# Autodesk Inventor assembly: TourniquetPCBV1_Updated
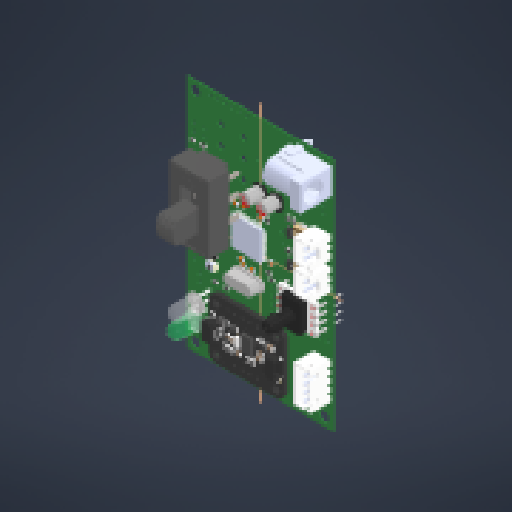
[picture p0: Inventor's stored thumbnail of the model, 512x512]
Saved by Autodesk Inventor 2026.2 (Build 302298010, 298A)
## iProperties
Company: Open CASCADE
Created: 2026-02-03
Part Number: TourniquetPCBV1_Updated
Description: Open CASCADE Model
Document SubType Name: Assembly
Designer: vckot
Authority: Unknown
Sending System: Open CASCADE 7.5
Preprocessor: Open CASCADE STEP processor 7.5
Title: Open CASCADE Shape Model
Author: Author
## Documents named in this file (48)
- C:\Users\jocel\OneDrive\Desktop\1 - IBEHS 5P06 CAPSTONE\capstone\CAD_files\Version_6\TourniquetPCBV1_Updated.iam
- C:\Users\jocel\OneDrive\Desktop\1 - IBEHS 5P06 CAPSTONE\capstone\CAD_files\Version_6\Board.iam
- C:\Users\jocel\OneDrive\Desktop\1 - IBEHS 5P06 CAPSTONE\capstone\CAD_files\Version_6\C16.iam
- C:\Users\jocel\OneDrive\Desktop\1 - IBEHS 5P06 CAPSTONE\capstone\CAD_files\Version_6\D7.iam
- C:\Users\jocel\OneDrive\Desktop\1 - IBEHS 5P06 CAPSTONE\capstone\CAD_files\Version_6\U5.iam
- C:\Users\jocel\OneDrive\Desktop\1 - IBEHS 5P06 CAPSTONE\capstone\CAD_files\Version_6\R21.iam
- C:\Users\jocel\OneDrive\Desktop\1 - IBEHS 5P06 CAPSTONE\capstone\CAD_files\Version_6\R20.iam
- C:\Users\jocel\OneDrive\Desktop\1 - IBEHS 5P06 CAPSTONE\capstone\CAD_files\Version_6\R19.iam
- C:\Users\jocel\OneDrive\Desktop\1 - IBEHS 5P06 CAPSTONE\capstone\CAD_files\Version_6\R2.iam
- C:\Users\jocel\OneDrive\Desktop\1 - IBEHS 5P06 CAPSTONE\capstone\CAD_files\Version_6\J6.iam
- C:\Users\jocel\OneDrive\Desktop\1 - IBEHS 5P06 CAPSTONE\capstone\CAD_files\Version_6\R9.iam
- C:\Users\jocel\OneDrive\Desktop\1 - IBEHS 5P06 CAPSTONE\capstone\CAD_files\Version_6\R7.iam
- C:\Users\jocel\OneDrive\Desktop\1 - IBEHS 5P06 CAPSTONE\capstone\CAD_files\Version_6\R5.iam
- C:\Users\jocel\OneDrive\Desktop\1 - IBEHS 5P06 CAPSTONE\capstone\CAD_files\Version_6\R3.iam
- C:\Users\jocel\OneDrive\Desktop\1 - IBEHS 5P06 CAPSTONE\capstone\CAD_files\Version_6\R11.iam
- C:\Users\jocel\OneDrive\Desktop\1 - IBEHS 5P06 CAPSTONE\capstone\CAD_files\Version_6\R10.iam
- C:\Users\jocel\OneDrive\Desktop\1 - IBEHS 5P06 CAPSTONE\capstone\CAD_files\Version_6\U4.iam
- C:\Users\jocel\OneDrive\Desktop\1 - IBEHS 5P06 CAPSTONE\capstone\CAD_files\Version_6\U1.iam
- C:\Users\jocel\OneDrive\Desktop\1 - IBEHS 5P06 CAPSTONE\capstone\CAD_files\Version_6\SW1.iam
- C:\Users\jocel\OneDrive\Desktop\1 - IBEHS 5P06 CAPSTONE\capstone\CAD_files\Version_6\R16.iam
- C:\Users\jocel\OneDrive\Desktop\1 - IBEHS 5P06 CAPSTONE\capstone\CAD_files\Version_6\R15.iam
- C:\Users\jocel\OneDrive\Desktop\1 - IBEHS 5P06 CAPSTONE\capstone\CAD_files\Version_6\R14.iam
- C:\Users\jocel\OneDrive\Desktop\1 - IBEHS 5P06 CAPSTONE\capstone\CAD_files\Version_6\R13.iam
- C:\Users\jocel\OneDrive\Desktop\1 - IBEHS 5P06 CAPSTONE\capstone\CAD_files\Version_6\R12.iam
- C:\Users\jocel\OneDrive\Desktop\1 - IBEHS 5P06 CAPSTONE\capstone\CAD_files\Version_6\R6.iam
- C:\Users\jocel\OneDrive\Desktop\1 - IBEHS 5P06 CAPSTONE\capstone\CAD_files\Version_6\R1.iam
- C:\Users\jocel\OneDrive\Desktop\1 - IBEHS 5P06 CAPSTONE\capstone\CAD_files\Version_6\Q3.iam
- C:\Users\jocel\OneDrive\Desktop\1 - IBEHS 5P06 CAPSTONE\capstone\CAD_files\Version_6\Q1.iam
- C:\Users\jocel\OneDrive\Desktop\1 - IBEHS 5P06 CAPSTONE\capstone\CAD_files\Version_6\O1.iam
- C:\Users\jocel\OneDrive\Desktop\1 - IBEHS 5P06 CAPSTONE\capstone\CAD_files\Version_6\J3.iam
- C:\Users\jocel\OneDrive\Desktop\1 - IBEHS 5P06 CAPSTONE\capstone\CAD_files\Version_6\J1.iam
- C:\Users\jocel\OneDrive\Desktop\1 - IBEHS 5P06 CAPSTONE\capstone\CAD_files\Version_6\FB1.iam
- C:\Users\jocel\OneDrive\Desktop\1 - IBEHS 5P06 CAPSTONE\capstone\CAD_files\Version_6\D3.iam
- C:\Users\jocel\OneDrive\Desktop\1 - IBEHS 5P06 CAPSTONE\capstone\CAD_files\Version_6\D1.iam
- C:\Users\jocel\OneDrive\Desktop\1 - IBEHS 5P06 CAPSTONE\capstone\CAD_files\Version_6\C15.iam
- C:\Users\jocel\OneDrive\Desktop\1 - IBEHS 5P06 CAPSTONE\capstone\CAD_files\Version_6\C12.iam
- C:\Users\jocel\OneDrive\Desktop\1 - IBEHS 5P06 CAPSTONE\capstone\CAD_files\Version_6\C11.iam
- C:\Users\jocel\OneDrive\Desktop\1 - IBEHS 5P06 CAPSTONE\capstone\CAD_files\Version_6\C10.iam
- C:\Users\jocel\OneDrive\Desktop\1 - IBEHS 5P06 CAPSTONE\capstone\CAD_files\Version_6\C9.iam
- C:\Users\jocel\OneDrive\Desktop\1 - IBEHS 5P06 CAPSTONE\capstone\CAD_files\Version_6\C8.iam
- C:\Users\jocel\OneDrive\Desktop\1 - IBEHS 5P06 CAPSTONE\capstone\CAD_files\Version_6\C7.iam
- C:\Users\jocel\OneDrive\Desktop\1 - IBEHS 5P06 CAPSTONE\capstone\CAD_files\Version_6\C6.iam
- C:\Users\jocel\OneDrive\Desktop\1 - IBEHS 5P06 CAPSTONE\capstone\CAD_files\Version_6\C5.iam
- C:\Users\jocel\OneDrive\Desktop\1 - IBEHS 5P06 CAPSTONE\capstone\CAD_files\Version_6\C4.iam
- C:\Users\jocel\OneDrive\Desktop\1 - IBEHS 5P06 CAPSTONE\capstone\CAD_files\Version_6\C3.iam
- C:\Users\jocel\OneDrive\Desktop\1 - IBEHS 5P06 CAPSTONE\capstone\CAD_files\Version_6\C2.iam
- C:\Users\jocel\OneDrive\Desktop\1 - IBEHS 5P06 CAPSTONE\capstone\CAD_files\Version_6\C1.iam
- C:\Users\jocel\OneDrive\Desktop\1 - IBEHS 5P06 CAPSTONE\capstone\CAD_files\Version_6\_.iam
## Components (47 placed, 47 different names)
1. Board_2 [sub-assembly] — Flush:1, Flush:2
2. C16_13 [sub-assembly]
3. D7_18 [sub-assembly]
4. U5_45 [sub-assembly]
5. R21_47 [sub-assembly]
6. R20_49 [sub-assembly]
7. R19_51 [sub-assembly]
8. R2_53 [sub-assembly]
9. J6_56 [sub-assembly]
10. R9_67 [sub-assembly]
11. R7_69 [sub-assembly]
12. R5_71 [sub-assembly]
13. R3_73 [sub-assembly]
14. R11_75 [sub-assembly]
15. R10_77 [sub-assembly]
16. U4_79 [sub-assembly]
17. U1_81 [sub-assembly]
18. SW1_83 [sub-assembly]
19. R16_85 [sub-assembly]
20. R15_87 [sub-assembly]
21. R14_89 [sub-assembly]
22. R13_91 [sub-assembly]
23. R12_93 [sub-assembly]
24. R6_95 [sub-assembly]
25. R1_97 [sub-assembly]
26. Q3_99 [sub-assembly]
27. Q1_101 [sub-assembly]
28. O1_103 [sub-assembly]
29. J3_106 [sub-assembly]
30. J1_108 [sub-assembly]
31. FB1_113 [sub-assembly]
32. D3_119 [sub-assembly]
33. D1_121 [sub-assembly]
34. C15_123 [sub-assembly]
35. C12_125 [sub-assembly]
36. C11_127 [sub-assembly]
37. C10_129 [sub-assembly]
38. C9_131 [sub-assembly]
39. C8_133 [sub-assembly]
40. C7_135 [sub-assembly]
41. C6_137 [sub-assembly]
42. C5_139 [sub-assembly]
43. C4_141 [sub-assembly]
44. C3_143 [sub-assembly]
45. C2_145 [sub-assembly]
46. C1_147 [sub-assembly]
47. __149 [sub-assembly]
## Relationships (2: Flush 2)
- Flush:1 (-40 mm): Board_2
- Flush:2 (-25 mm): Board_2
## Named parameters: Finish2_Area = 1.40949
note: some values were not read from the file. Shown as the stored number, unit unknown: "Finish2_Area".
